# Autodesk Inventor assembly: Camera Mount
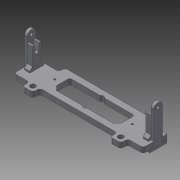
[picture p0: Inventor's stored thumbnail of the model, 180x180]
Saved by Autodesk Inventor 2015 (Build 190159000, 159)
## iProperties
Created: 2015-07-21
Part Number: Camera Mount
Document SubType Name: Assembly
Designer: JR
Author: JR
## Documents named in this file (4)
- F:\OpenROV\2.8\Electronics Tube\Forward\Camera Mount.iam
- F:\OpenROV\2.8\Electronics Tube\Forward\camera_mount_v1.ipt
- F:\OpenROV\2.8\Electronics Tube\Forward\arm3mm.ipt
- F:\OpenROV\2.8\Electronics Tube\Forward\arm 6mm.ipt
## Components (5 placed, 3 different names)
1. camera_mount_v1:1 — Mate:1, Flush:1, Mate:2, Mate:3, Flush:2, Mate:4, Flush:4, Flush:6
2. arm3mm:1 — Mate:6, Flush:5, Flush:6
3. arm3mm:2 — Mate:5, Flush:3, Flush:4
4. arm 6mm:1 — Mate:1, Flush:1, Mate:2, Mate:6, Flush:5
5. arm 6mm:2 — Mate:3, Flush:2, Mate:4, Mate:5, Flush:3
## Relationships (12: Mate 6, Flush 6)
- Mate:1: camera_mount_v1:1 ↔ arm 6mm:1
- Flush:1: camera_mount_v1:1 ↔ arm 6mm:1
- Mate:2: camera_mount_v1:1 ↔ arm 6mm:1
- Mate:3: camera_mount_v1:1 ↔ arm 6mm:2
- Flush:2: camera_mount_v1:1 ↔ arm 6mm:2
- Mate:4: camera_mount_v1:1 ↔ arm 6mm:2
- Mate:5: arm3mm:2 ↔ arm 6mm:2
- Flush:3: arm3mm:2 ↔ arm 6mm:2
- Flush:4: camera_mount_v1:1 ↔ arm3mm:2
- Mate:6: arm3mm:1 ↔ arm 6mm:1
- Flush:5: arm3mm:1 ↔ arm 6mm:1
- Flush:6: camera_mount_v1:1 ↔ arm3mm:1
